# Autodesk Inventor assembly: elbowassembly
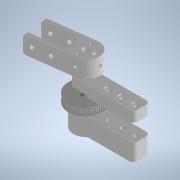
[picture p0: Inventor's stored thumbnail of the model, 180x180]
Saved by Autodesk Inventor 2022 (Build 260153000, 153)
## iProperties
Created: 2022-02-22
Part Number: elbowassembly
Document SubType Name: Assembly
Designer: JK
Author: JK
## Documents named in this file (6)
- C:\Users\JK\Documents\Inventor\ScaraNema\SCARA-3DP\Parts\Elbow\Elbow assembly.iam
- C:\Users\JK\Documents\Inventor\ScaraNema\SCARA-3DP\Parts\Elbow\GT260T.ipt
- C:\Users\JK\Documents\Inventor\ScaraNema\SCARA-3DP\Parts\Elbow\top support.ipt
- C:\Users\JK\Documents\Inventor\ScaraNema\SCARA-3DP\Parts\Elbow\bottomsupport.ipt
- C:\Users\JK\Documents\Inventor\ScaraNema\SCARA-3DP\Parts\Elbow\Bearing.ipt
- C:\Users\JK\Documents\Inventor\ScaraNema\SCARA-3DP\Parts\Elbow\Soporte antebrazo.ipt
## Components (6 placed, 5 different names)
1. GT260T:1 — Coincidencia:21, Coincidencia:22, Coincidencia:23, Coincidencia:24
2. bottomsupport:1 — Coincidencia:19, Coincidencia:20, Coincidencia:24
3. Bearing:1 — Coincidencia:19, Coincidencia:20, Coincidencia:21
4. Bearing:2 — Coincidencia:22, Coincidencia:23, Coincidencia:26
5. top support:1 — Coincidencia:26, Coincidencia:27
6. Soporte antebrazo:1 — Coincidencia:27
## Relationships (8: Mate 8)
- Coincidencia:19 [Mate]: bottomsupport:1 ↔ Bearing:1
- Coincidencia:20 [Mate]: bottomsupport:1 ↔ Bearing:1
- Coincidencia:21 [Mate]: GT260T:1 ↔ Bearing:1
- Coincidencia:22 [Mate]: GT260T:1 ↔ Bearing:2
- Coincidencia:23 [Mate] (1 mm): GT260T:1 ↔ Bearing:2
- Coincidencia:24 [Mate] (7 mm): GT260T:1 ↔ bottomsupport:1
- Coincidencia:26 [Mate]: Bearing:2 ↔ top support:1
- Coincidencia:27 [Mate]: top support:1 ↔ Soporte antebrazo:1
